# Autodesk Inventor assembly: 機体
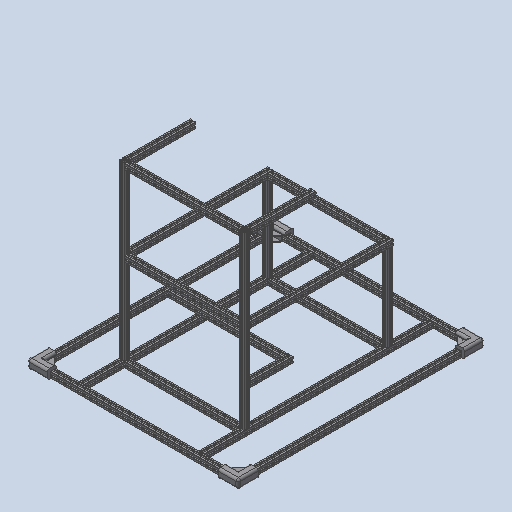
[picture p0: Inventor's stored thumbnail of the model, 512x512]
Saved by Autodesk Inventor 2022 (Build 260153000, 153)
## iProperties
Part Number: 機体
Material: 一般
Document SubType Name: Assembly
Designer: highs
Author: highs
## Documents named in this file (11)
- D:\Navitoon\フレーム.iam
- D:\Navitoon\高剛性フレーム1.ipt
- D:\Navitoon\高剛性フレーム2.ipt
- D:\Navitoon\高剛性フレーム3.ipt
- D:\Navitoon\高剛性フレーム4.ipt
- D:\Navitoon\高剛性フレーム5.ipt
- D:\Navitoon\高剛性フレーム6.ipt
- D:\Navitoon\クッション.ipt
- D:\Navitoon\ブラケット2.ipt
- D:\Navitoon\高剛性フレーム8.ipt
- D:\Navitoon\高剛性フレーム9.ipt
## Components (30 placed, 10 different names)
1. 高剛性フレーム1:1 — メイト:1, フラッシュ:1, フラッシュ:2, フラッシュ:5, フラッシュ:6, メイト:3, メイト:6, メイト:36, メイト:41, メイト:44, メイト:47, フラッシュ:39
2. 高剛性フレーム2:1 — メイト:8, フラッシュ:9, フラッシュ:11, メイト:13, フラッシュ:17, フラッシュ:18
3. 高剛性フレーム3:1 — メイト:1, フラッシュ:1, フラッシュ:2, フラッシュ:3, メイト:2, フラッシュ:4, フラッシュ:26, メイト:34, メイト:37, メイト:43, フラッシュ:37, メイト:45, フラッシュ:38
4. 高剛性フレーム1:2 — フラッシュ:3, メイト:2, フラッシュ:4, メイト:7, メイト:35, メイト:38, メイト:42, メイト:48
5. 高剛性フレーム3:2 — フラッシュ:5, フラッシュ:6, メイト:3, フラッシュ:7, フラッシュ:8, メイト:4, メイト:5, メイト:30, メイト:31, メイト:32, メイト:33, メイト:39, メイト:40, メイト:46, メイト:49, フラッシュ:40
6. 高剛性フレーム1:3 — フラッシュ:7, メイト:4, メイト:6, フラッシュ:10, メイト:9, メイト:18
7. 高剛性フレーム1:4 — フラッシュ:8, メイト:5, メイト:7, メイト:8, フラッシュ:9, メイト:16, メイト:26, メイト:27, フラッシュ:32, フラッシュ:33, メイト:55
8. 高剛性フレーム4:3 — フラッシュ:16, メイト:14, メイト:17, フラッシュ:20, フラッシュ:21, メイト:29, フラッシュ:43
9. 高剛性フレーム2:2 — フラッシュ:10, メイト:9, フラッシュ:11, フラッシュ:16, メイト:14, フラッシュ:21, フラッシュ:34
10. 高剛性フレーム5:3 — メイト:17, メイト:18, フラッシュ:20, メイト:24, フラッシュ:30, メイト:25, フラッシュ:31, メイト:50, フラッシュ:47, メイト:53, フラッシュ:49
11. 高剛性フレーム4:4 — メイト:13, フラッシュ:17, フラッシュ:18, メイト:15, フラッシュ:19, フラッシュ:35, フラッシュ:36
12. 高剛性フレーム5:4 — メイト:15, メイト:16, フラッシュ:19, フラッシュ:26, フラッシュ:41, フラッシュ:42, メイト:51, フラッシュ:46, フラッシュ:48, メイト:52
13. 高剛性フレーム6:1 — メイト:25, フラッシュ:31, フラッシュ:42, フラッシュ:44, フラッシュ:45
14. 高剛性フレーム6:2 — メイト:24, フラッシュ:30, フラッシュ:43
15. 高剛性フレーム6:3 — フラッシュ:35, メイト:29, フラッシュ:36
16. 高剛性フレーム6:4 — メイト:27, フラッシュ:33, フラッシュ:34
17. 高剛性フレーム6:5 — メイト:26, フラッシュ:32, フラッシュ:41
18. クッション:1 — メイト:31, メイト:38, メイト:39
19. クッション:2 — メイト:30, メイト:40, メイト:41
20. クッション:3 — メイト:33, メイト:36, メイト:37
21. クッション:4 — メイト:32, メイト:34, メイト:35
22. ブラケット2:1 — メイト:42, メイト:43, フラッシュ:37
23. ブラケット2:2 — メイト:46, メイト:47, フラッシュ:39
24. ブラケット2:3 — メイト:48, メイト:49, フラッシュ:40
25. ブラケット2:4 — メイト:44, メイト:45, フラッシュ:38
26. 高剛性フレーム8:1 — フラッシュ:44, メイト:50, フラッシュ:47
27. 高剛性フレーム8:2 — フラッシュ:45, メイト:51, フラッシュ:46
28. 高剛性フレーム9:1 — フラッシュ:48, メイト:52, フラッシュ:50, フラッシュ:51, メイト:54, フラッシュ:52, メイト:55
29. 高剛性フレーム9:2 — メイト:53, フラッシュ:49, フラッシュ:50
30. 高剛性フレーム6:6 — フラッシュ:51, メイト:54, フラッシュ:52
## Relationships (87: Mate 46, Flush 41)
- メイト:1 [Mate]: 高剛性フレーム1:1 ↔ 高剛性フレーム3:1
- フラッシュ:1 [Flush]: 高剛性フレーム1:1 ↔ 高剛性フレーム3:1
- フラッシュ:2 [Flush]: 高剛性フレーム1:1 ↔ 高剛性フレーム3:1
- フラッシュ:3 [Flush]: 高剛性フレーム3:1 ↔ 高剛性フレーム1:2
- メイト:2 [Mate]: 高剛性フレーム3:1 ↔ 高剛性フレーム1:2
- フラッシュ:4 [Flush]: 高剛性フレーム3:1 ↔ 高剛性フレーム1:2
- フラッシュ:5 [Flush]: 高剛性フレーム1:1 ↔ 高剛性フレーム3:2
- フラッシュ:6 [Flush]: 高剛性フレーム1:1 ↔ 高剛性フレーム3:2
- メイト:3 [Mate]: 高剛性フレーム1:1 ↔ 高剛性フレーム3:2
- フラッシュ:7 [Flush]: 高剛性フレーム3:2 ↔ 高剛性フレーム1:3
- フラッシュ:8 [Flush]: 高剛性フレーム3:2 ↔ 高剛性フレーム1:4
- メイト:4 [Mate]: 高剛性フレーム3:2 ↔ 高剛性フレーム1:3
- メイト:5 [Mate]: 高剛性フレーム3:2 ↔ 高剛性フレーム1:4
- メイト:6 [Mate] (118 mm): 高剛性フレーム1:1 ↔ 高剛性フレーム1:3
- メイト:7 [Mate] (118 mm): 高剛性フレーム1:2 ↔ 高剛性フレーム1:4
- メイト:8 [Mate]: 高剛性フレーム2:1 ↔ 高剛性フレーム1:4
- フラッシュ:9 [Flush]: 高剛性フレーム2:1 ↔ 高剛性フレーム1:4
- フラッシュ:10 [Flush]: 高剛性フレーム1:3 ↔ 高剛性フレーム2:2
- メイト:9 [Mate]: 高剛性フレーム1:3 ↔ 高剛性フレーム2:2
- フラッシュ:11 [Flush]: 高剛性フレーム2:1 ↔ 高剛性フレーム2:2
- フラッシュ:16 [Flush]: 高剛性フレーム4:3 ↔ 高剛性フレーム2:2
- メイト:13 [Mate]: 高剛性フレーム2:1 ↔ 高剛性フレーム4:4
- フラッシュ:17 [Flush]: 高剛性フレーム2:1 ↔ 高剛性フレーム4:4
- フラッシュ:18 [Flush]: 高剛性フレーム2:1 ↔ 高剛性フレーム4:4
- メイト:14 [Mate]: 高剛性フレーム4:3 ↔ 高剛性フレーム2:2
- メイト:15 [Mate]: 高剛性フレーム4:4 ↔ 高剛性フレーム5:4
- メイト:16 [Mate]: 高剛性フレーム1:4 ↔ 高剛性フレーム5:4
- メイト:17 [Mate]: 高剛性フレーム4:3 ↔ 高剛性フレーム5:3
- メイト:18 [Mate]: 高剛性フレーム1:3 ↔ 高剛性フレーム5:3
- フラッシュ:19 [Flush]: 高剛性フレーム4:4 ↔ 高剛性フレーム5:4
- フラッシュ:20 [Flush]: 高剛性フレーム4:3 ↔ 高剛性フレーム5:3
- フラッシュ:21 [Flush]: 高剛性フレーム4:3 ↔ 高剛性フレーム2:2
- フラッシュ:26 [Flush] (160 mm): 高剛性フレーム3:1 ↔ 高剛性フレーム5:4
- メイト:24 [Mate]: 高剛性フレーム5:3 ↔ 高剛性フレーム6:2
- フラッシュ:30 [Flush]: 高剛性フレーム5:3 ↔ 高剛性フレーム6:2
- メイト:25 [Mate]: 高剛性フレーム5:3 ↔ 高剛性フレーム6:1
- フラッシュ:31 [Flush]: 高剛性フレーム5:3 ↔ 高剛性フレーム6:1
- メイト:26 [Mate]: 高剛性フレーム1:4 ↔ 高剛性フレーム6:5
- メイト:27 [Mate]: 高剛性フレーム1:4 ↔ 高剛性フレーム6:4
- フラッシュ:32 [Flush]: 高剛性フレーム1:4 ↔ 高剛性フレーム6:5
- フラッシュ:33 [Flush]: 高剛性フレーム1:4 ↔ 高剛性フレーム6:4
- フラッシュ:34 [Flush]: 高剛性フレーム2:2 ↔ 高剛性フレーム6:4
- フラッシュ:35 [Flush]: 高剛性フレーム4:4 ↔ 高剛性フレーム6:3
- メイト:29 [Mate]: 高剛性フレーム4:3 ↔ 高剛性フレーム6:3
- フラッシュ:36 [Flush]: 高剛性フレーム4:4 ↔ 高剛性フレーム6:3
- メイト:30 [Mate]: 高剛性フレーム3:2 ↔ クッション:2
- メイト:31 [Mate]: 高剛性フレーム3:2 ↔ クッション:1
- メイト:32 [Mate]: 高剛性フレーム3:2 ↔ クッション:4
- メイト:33 [Mate]: 高剛性フレーム3:2 ↔ クッション:3
- メイト:34 [Mate]: 高剛性フレーム3:1 ↔ クッション:4
- メイト:35 [Mate]: 高剛性フレーム1:2 ↔ クッション:4
- メイト:36 [Mate]: 高剛性フレーム1:1 ↔ クッション:3
- メイト:37 [Mate]: 高剛性フレーム3:1 ↔ クッション:3
- メイト:38 [Mate]: 高剛性フレーム1:2 ↔ クッション:1
- メイト:39 [Mate]: 高剛性フレーム3:2 ↔ クッション:1
- メイト:40 [Mate]: 高剛性フレーム3:2 ↔ クッション:2
- メイト:41 [Mate]: 高剛性フレーム1:1 ↔ クッション:2
- メイト:42 [Mate]: 高剛性フレーム1:2 ↔ ブラケット2:1
- メイト:43 [Mate]: 高剛性フレーム3:1 ↔ ブラケット2:1
- フラッシュ:37 [Flush]: 高剛性フレーム3:1 ↔ ブラケット2:1
- メイト:44 [Mate]: 高剛性フレーム1:1 ↔ ブラケット2:4
- メイト:45 [Mate]: 高剛性フレーム3:1 ↔ ブラケット2:4
- フラッシュ:38 [Flush]: 高剛性フレーム3:1 ↔ ブラケット2:4
- メイト:46 [Mate]: 高剛性フレーム3:2 ↔ ブラケット2:2
- メイト:47 [Mate]: 高剛性フレーム1:1 ↔ ブラケット2:2
- フラッシュ:39 [Flush]: 高剛性フレーム1:1 ↔ ブラケット2:2
- メイト:48 [Mate]: 高剛性フレーム1:2 ↔ ブラケット2:3
- メイト:49 [Mate]: 高剛性フレーム3:2 ↔ ブラケット2:3
- フラッシュ:40 [Flush]: 高剛性フレーム3:2 ↔ ブラケット2:3
- フラッシュ:41 [Flush]: 高剛性フレーム5:4 ↔ 高剛性フレーム6:5
- フラッシュ:42 [Flush]: 高剛性フレーム5:4 ↔ 高剛性フレーム6:1
- フラッシュ:43 [Flush]: 高剛性フレーム4:3 ↔ 高剛性フレーム6:2
- フラッシュ:44 [Flush]: 高剛性フレーム6:1 ↔ 高剛性フレーム8:1
- フラッシュ:45 [Flush]: 高剛性フレーム6:1 ↔ 高剛性フレーム8:2
- メイト:50 [Mate]: 高剛性フレーム5:3 ↔ 高剛性フレーム8:1
- メイト:51 [Mate]: 高剛性フレーム5:4 ↔ 高剛性フレーム8:2
- フラッシュ:46 [Flush]: 高剛性フレーム5:4 ↔ 高剛性フレーム8:2
- フラッシュ:47 [Flush]: 高剛性フレーム5:3 ↔ 高剛性フレーム8:1
- フラッシュ:48 [Flush]: 高剛性フレーム5:4 ↔ 高剛性フレーム9:1
- メイト:52 [Mate]: 高剛性フレーム5:4 ↔ 高剛性フレーム9:1
- メイト:53 [Mate]: 高剛性フレーム5:3 ↔ 高剛性フレーム9:2
- フラッシュ:49 [Flush]: 高剛性フレーム5:3 ↔ 高剛性フレーム9:2
- フラッシュ:50 [Flush]: 高剛性フレーム9:1 ↔ 高剛性フレーム9:2
- フラッシュ:51 [Flush]: 高剛性フレーム9:1 ↔ 高剛性フレーム6:6
- メイト:54 [Mate]: 高剛性フレーム9:1 ↔ 高剛性フレーム6:6
- フラッシュ:52 [Flush]: 高剛性フレーム9:1 ↔ 高剛性フレーム6:6
- メイト:55 [Mate] (120 mm): 高剛性フレーム1:4 ↔ 高剛性フレーム9:1
